# Autodesk Inventor assembly: one roller asmb
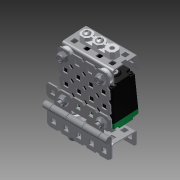
[picture p0: Inventor's stored thumbnail of the model, 180x180]
Saved by Autodesk Inventor 2014 SP1 (Build 180222100, 222)
## iProperties
Created: 2014-03-20
Part Number: one roller asmb
Document SubType Name: Assembly
Designer: Ryan
Author: Ryan
## Documents named in this file (16)
- C:\Users\Ryan\Desktop\sw\toss up 5th A bot\intake\one roller asmb.iam
- C:\Users\Ryan\Desktop\sw\lib\Aperture VEX CAD Library\Metal\C Channel\2 x 5.ipt
- C:\Users\Ryan\Desktop\sw\lib\Aperture VEX CAD Library\Metal\C Channel\2 x 4.ipt
- C:\Users\Ryan\Desktop\sw\lib\Aperture VEX CAD Library\Metal\Plate\4 x 4.ipt
- C:\Users\Ryan\Desktop\sw\lib\Aperture VEX CAD Library\Metal\vex hinge\hinge.iam
- C:\Users\Ryan\Desktop\sw\lib\Aperture VEX CAD Library\Hardware\8-32\8-32_.375.ipt
- C:\Users\Ryan\Desktop\sw\lib\Aperture VEX CAD Library\Hardware\8-32\8-32 nylock.ipt
- C:\Users\Ryan\Desktop\sw\lib\Aperture VEX CAD Library\Spacers\SPACER-0500-0125.ipt
- C:\Users\Ryan\Desktop\sw\lib\Aperture VEX CAD Library\Bearing Blocks\Bearing Block.ipt
- C:\Users\Ryan\Desktop\sw\lib\Aperture VEX CAD Library\Motors\2-Wire Motor 393-Without Wire.iam
- C:\Users\Ryan\Desktop\sw\lib\Aperture VEX CAD Library\Hardware\6-32\6-32_.500.ipt
- C:\Users\Ryan\Desktop\sw\lib\Aperture VEX CAD Library\Spacers\thin\SPACER-0320-0500.ipt
- C:\Users\Ryan\Desktop\sw\lib\Aperture VEX CAD Library\Hardware\8-32\8-32_.875.ipt
- C:\Users\Ryan\Desktop\sw\lib\Aperture VEX CAD Library\Spacers\thin\SPACER-0320-0125.ipt
- C:\Users\Ryan\Desktop\sw\lib\Aperture VEX CAD Library\Spacers\thin\SPACER-0320-0375.ipt
- C:\Users\Ryan\Desktop\sw\lib\Aperture VEX CAD Library\Hardware\8-32\8-23_.750.ipt
## Components (30 placed, 15 different names)
1. 2 x 5:1 — Flush:5, Flush:6, Mate:2, Mate:96, Mate:97, Mate:98, Mate:99, Mate:107, Mate:108, Mate:109, Mate:110, Mate:112, Mate:114, Mate:115, Mate:119
2. 2 x 4:1 — Flush:1, Flush:2, Mate:9, Mate:10, Mate:11, Mate:12, Mate:13, Mate:14, Mate:27, Mate:52, Mate:53, Mate:54, Mate:55, Mate:87
3. 4 x 4:1 — Flush:1, Flush:2, Mate:1, Flush:3, Flush:4, Mate:3, Mate:4, Mate:5, Mate:6, Mate:7, Mate:8, Mate:16, Mate:22, Mate:23, Mate:26
4. hinge:1 [sub-assembly] — Mate:1, Flush:3, Flush:4, Flush:5, Flush:6, Mate:2, Mate:20, Mate:21
5. 8-32_.375:1 — Mate:3, Mate:4, Mate:5, Mate:17
6. 8-32_.375:2 — Mate:6, Mate:7, Mate:8, Mate:18
7. 8-32_.375:3 — Mate:9, Mate:10, Mate:11, Mate:15, Mate:24
8. 8-32_.375:4 — Mate:12, Mate:13, Mate:14, Mate:19, Mate:25
9. 8-32 nylock:1 — Mate:15, Mate:16
10. 8-32 nylock:2 — Mate:18, Mate:21
11. 8-32 nylock:3 — Mate:19, Mate:22
12. 8-32 nylock:4 — Mate:17, Mate:20
13. SPACER-0500-0125:1 — Mate:23, Mate:24
14. SPACER-0500-0125:2 — Mate:25, Mate:26, Mate:27
15. Bearing Block:1 — Mate:52, Mate:53, Mate:54, Mate:55, Mate:88, Mate:89, Mate:90, Mate:91, Mate:92
16. 2-Wire Motor 393-Without Wire:1 [sub-assembly] — Mate:87, Mate:88, Mate:89
17. 6-32_.500:1 — Mate:90, Flush:7, Mate:92
18. 6-32_.500:2 — Mate:91, Flush:7
19. SPACER-0500-0125:3 — Mate:93, Mate:94, Mate:98
20. SPACER-0320-0500:1 — Mate:95, Mate:99, Mate:100
21. 8-32_.875:1 — Mate:93, Mate:94, Mate:95, Mate:96, Mate:97, Mate:101
22. 8-32 nylock:8 — Mate:100, Mate:101
23. SPACER-0500-0125:4 — Mate:109
24. SPACER-0320-0500:2 — Mate:110
25. 8-32_.875:2 — Mate:107, Mate:108
26. 8-32 nylock:9
27. SPACER-0320-0125:1 — Mate:111, Mate:113, Mate:117
28. SPACER-0320-0375:1 — Mate:111, Mate:112, Mate:113, Mate:114, Mate:115, Mate:116
29. 8-23_.750:1 — Mate:116, Mate:117, Mate:118
30. 8-32 nylock:10 — Mate:118, Mate:119
## Relationships (71: Mate 64, Flush 7)
- Flush:1: 2 x 4:1 ↔ 4 x 4:1
- Flush:2: 2 x 4:1 ↔ 4 x 4:1
- Mate:1: 4 x 4:1 ↔ hinge:1
- Flush:3: 4 x 4:1 ↔ hinge:1
- Flush:4: 4 x 4:1 ↔ hinge:1
- Flush:5: 2 x 5:1 ↔ hinge:1
- Flush:6: 2 x 5:1 ↔ hinge:1
- Mate:2: 2 x 5:1 ↔ hinge:1
- Mate:3 (2.3114 mm): 4 x 4:1 ↔ 8-32_.375:1
- Mate:4 (2.3114 mm): 4 x 4:1 ↔ 8-32_.375:1
- Mate:5: 4 x 4:1 ↔ 8-32_.375:1
- Mate:6 (2.3114 mm): 4 x 4:1 ↔ 8-32_.375:2
- Mate:7 (2.3114 mm): 4 x 4:1 ↔ 8-32_.375:2
- Mate:8: 4 x 4:1 ↔ 8-32_.375:2
- Mate:9: 2 x 4:1 ↔ 8-32_.375:3
- Mate:10 (2.3114 mm): 2 x 4:1 ↔ 8-32_.375:3
- Mate:11 (2.3114 mm): 2 x 4:1 ↔ 8-32_.375:3
- Mate:12 (2.3114 mm): 2 x 4:1 ↔ 8-32_.375:4
- Mate:13 (2.3114 mm): 2 x 4:1 ↔ 8-32_.375:4
- Mate:14: 2 x 4:1 ↔ 8-32_.375:4
- Mate:15: 8-32_.375:3 ↔ 8-32 nylock:1
- Mate:16: 4 x 4:1 ↔ 8-32 nylock:1
- Mate:17: 8-32_.375:1 ↔ 8-32 nylock:4
- Mate:18: 8-32_.375:2 ↔ 8-32 nylock:2
- Mate:19: 8-32_.375:4 ↔ 8-32 nylock:3
- Mate:20: hinge:1 ↔ 8-32 nylock:4
- Mate:21: hinge:1 ↔ 8-32 nylock:2
- Mate:22: 4 x 4:1 ↔ 8-32 nylock:3
- Mate:23: 4 x 4:1 ↔ SPACER-0500-0125:1
- Mate:24: 8-32_.375:3 ↔ SPACER-0500-0125:1
- Mate:25: 8-32_.375:4 ↔ SPACER-0500-0125:2
- Mate:26: 4 x 4:1 ↔ SPACER-0500-0125:2
- Mate:27: 2 x 4:1 ↔ SPACER-0500-0125:2
- Mate:52: 2 x 4:1 ↔ Bearing Block:1
- Mate:53 (2.3114 mm): 2 x 4:1 ↔ Bearing Block:1
- Mate:54 (2.3114 mm): 2 x 4:1 ↔ Bearing Block:1
- Mate:55 (2.3114 mm): 2 x 4:1 ↔ Bearing Block:1
- Mate:87: 2 x 4:1 ↔ 2-Wire Motor 393-Without Wire:1
- Mate:88: Bearing Block:1 ↔ 2-Wire Motor 393-Without Wire:1
- Mate:89: Bearing Block:1 ↔ 2-Wire Motor 393-Without Wire:1
- Mate:90: Bearing Block:1 ↔ 6-32_.500:1
- Mate:91: Bearing Block:1 ↔ 6-32_.500:2
- Flush:7: 6-32_.500:1 ↔ 6-32_.500:2
- Mate:92: Bearing Block:1 ↔ 6-32_.500:1
- Mate:93: SPACER-0500-0125:3 ↔ 8-32_.875:1
- Mate:94: SPACER-0500-0125:3 ↔ 8-32_.875:1
- Mate:95: SPACER-0320-0500:1 ↔ 8-32_.875:1
- Mate:96 (2.3114 mm): 2 x 5:1 ↔ 8-32_.875:1
- Mate:97 (2.3114 mm): 2 x 5:1 ↔ 8-32_.875:1
- Mate:98: 2 x 5:1 ↔ SPACER-0500-0125:3
- Mate:99: 2 x 5:1 ↔ SPACER-0320-0500:1
- Mate:100 (1.1684 mm): SPACER-0320-0500:1 ↔ 8-32 nylock:8
- Mate:101: 8-32_.875:1 ↔ 8-32 nylock:8
- [Mate]: SPACER-0500-0125:4 ↔ 8-32_.875:2
- [Mate]: SPACER-0500-0125:4 ↔ 8-32_.875:2
- [Mate]: SPACER-0320-0500:2 ↔ 8-32_.875:2
- [Mate] (1.1684 mm): SPACER-0320-0500:2 ↔ 8-32 nylock:9
- [Mate]: 8-32_.875:2 ↔ 8-32 nylock:9
- Mate:107 (2.3114 mm): 2 x 5:1 ↔ 8-32_.875:2
- Mate:108 (2.3114 mm): 2 x 5:1 ↔ 8-32_.875:2
- Mate:109: 2 x 5:1 ↔ SPACER-0500-0125:4
- Mate:110: 2 x 5:1 ↔ SPACER-0320-0500:2
- Mate:111: SPACER-0320-0125:1 ↔ SPACER-0320-0375:1
- Mate:112: 2 x 5:1 ↔ SPACER-0320-0375:1
- Mate:113: SPACER-0320-0125:1 ↔ SPACER-0320-0375:1
- Mate:114 (2.3114 mm): 2 x 5:1 ↔ SPACER-0320-0375:1
- Mate:115 (2.3114 mm): 2 x 5:1 ↔ SPACER-0320-0375:1
- Mate:116: SPACER-0320-0375:1 ↔ 8-23_.750:1
- Mate:117: SPACER-0320-0125:1 ↔ 8-23_.750:1
- Mate:118: 8-23_.750:1 ↔ 8-32 nylock:10
- Mate:119: 2 x 5:1 ↔ 8-32 nylock:10
## Named parameters: q = 2.3114 mm, d114_d105 = 0 mm, d115_d106 = 0 mm, d116_d107 = 0 mm, d117_d112 = 1.1684 mm, d118_d113 = 0 mm
